# Autodesk Inventor assembly: spinning thing
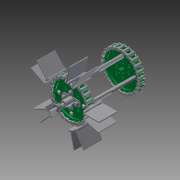
[picture p0: Inventor's stored thumbnail of the model, 180x180]
Saved by Autodesk Inventor 2014 SP1 (Build 180222100, 222)
## iProperties
Created: 2014-02-27
Part Number: spinning thing
Document SubType Name: Assembly
Designer: Ryan
Author: Ryan
## Documents named in this file (14)
- C:\Users\Ryan\Desktop\sw\toss up 5th A bot\intake\spinning thing.iam
- C:\Users\Ryan\Desktop\sw\lib\Aperture VEX CAD Library\Sprockets\HS Sprockets\High strength Chain Link.ipt
- C:\Users\Ryan\Desktop\sw\lib\Aperture VEX CAD Library\Tank Tread\flap-Link.ipt
- C:\Users\Ryan\Desktop\sw\lib\Aperture VEX CAD Library\Tank Tread\flaps\Conveyor-Fin-Tall.ipt
- C:\Users\Ryan\Desktop\sw\lib\Aperture VEX CAD Library\Sprockets\green\High Strength 24-Tooth Sprocket.ipt
- C:\Users\Ryan\Desktop\sw\lib\Aperture VEX CAD Library\Spacers\SPACER-0500-0375.ipt
- C:\Users\Ryan\Desktop\sw\lib\Aperture VEX CAD Library\Standoffs\BEAM-2000.ipt
- C:\Users\Ryan\Desktop\sw\lib\Aperture VEX CAD Library\Hardware\8-32\8-32_.375.ipt
- C:\Users\Ryan\Desktop\sw\lib\Aperture VEX CAD Library\Shaft\3 inch Shaft.ipt
- C:\Users\Ryan\Desktop\sw\lib\Aperture VEX CAD Library\Hardware\Shaft Collar.ipt
- C:\Users\Ryan\Desktop\sw\lib\Aperture VEX CAD Library\Sprockets\green\High Strength 24-Tooth Sprocket no knobs.ipt
- C:\Users\Ryan\Desktop\sw\lib\Aperture VEX CAD Library\Metal\Gussets\Lockbar.ipt
- C:\Users\Ryan\Desktop\sw\lib\Aperture VEX CAD Library\Hardware\8-32\8-32 nylock.ipt
- C:\Users\Ryan\Desktop\sw\lib\Aperture VEX CAD Library\Spacers\SPACER-0500-0250.ipt
## Components (91 placed, 13 different names)
1. High Strength 24-Tooth Sprocket no knobs:1 — Mate:15, Mate:16, Mate:17, Tangent:3, Mate:20, Mate:21, Mate:35, Mate:36, Flush:40, Mate:39, Mate:40, Mate:46, Mate:59, Mate:60, Tangent:8, Mate:66, Mate:67, Mate:69, Mate:70, Mate:78, Mate:79, Mate:80
2. SPACER-0500-0375:1 — Mate:18, Mate:43, Mate:44, Mate:73, Mate:84, Mate:85
3. High Strength 24-Tooth Sprocket:2 — Mate:25, Mate:26, Mate:33, Mate:34, Mate:37, Mate:38, Mate:18, Mate:72, Mate:48, Mate:61, Mate:62
4. 3 inch Shaft:1 — Flush:40, Mate:39, Mate:40, Mate:64, Mate:65, Mate:74
5. Shaft Collar:1 — Mate:71, Mate:72, Mate:73, Mate:74
6. Shaft Collar:2 — Mate:43, Mate:44
7. High strength Chain Link:35 — Mate:60
8. flap-Link:9 — Tangent:8
9. Conveyor-Fin-Tall:9
10. High strength Chain Link:36 — Flush:63, Mate:59, Mate:61
11. flap-Link:10 — Mate:62
12. Conveyor-Fin-Tall:10
13. Lockbar:1 — Mate:64, Mate:65, Mate:66, Mate:82, Mate:83
14. Lockbar:2 — Mate:67, Mate:69, Mate:70, Mate:71, Mate:75, Mate:76
15. SPACER-0500-0250:1 — Mate:83, Mate:84, Mate:85
16. flap-Link:2 — Mate:7, Mate:8, Mate:9, Mate:10, Flush:7, Mate:48
17. Conveyor-Fin-Tall:2 — Flush:8, Mate:11, Mate:12
18. flap-Link:1 — Mate:1, Mate:2, Mate:7, Flush:8, Mate:11, Mate:12, Tangent:3
19. High strength Chain Link:1 — Mate:1, Mate:2, Mate:8, Mate:13, Mate:14, Mate:17
20. High strength Chain Link:2 — Mate:13, Mate:14, Mate:15, Mate:16, Mate:45, Mate:47, Flush:63
21. High strength Chain Link:25 — Mate:45, Mate:46, Mate:47
22. Conveyor-Fin-Tall:1 — Mate:9, Mate:10, Flush:7
23. flap-Link:3
24. Conveyor-Fin-Tall:3
25. flap-Link:4
26. High strength Chain Link:26
27. High strength Chain Link:27
28. High strength Chain Link:28
29. Conveyor-Fin-Tall:6
30. flap-Link:5
31. Conveyor-Fin-Tall:4
32. flap-Link:6
33. High strength Chain Link:29
34. High strength Chain Link:30
35. High strength Chain Link:31
36. Conveyor-Fin-Tall:7
37. flap-Link:7
38. Conveyor-Fin-Tall:5
39. flap-Link:8
40. High strength Chain Link:32
41. High strength Chain Link:33
42. High strength Chain Link:34
43. Conveyor-Fin-Tall:8
44. 8-32_.375:11 — Mate:79, Mate:80, Mate:81
45. 8-32_.375:10 — Mate:75, Mate:76, Mate:77
46. 8-32 nylock:2 — Mate:81, Mate:82
47. 8-32 nylock:1 — Mate:77, Mate:78
48. 8-32_.375:12
49. 8-32_.375:13
50. 8-32 nylock:3
51. 8-32 nylock:4
52. BEAM-2000:1 — Mate:20, Mate:21, Mate:22, Mate:23
53. BEAM-2000:2 — Mate:22, Mate:23, Mate:25, Mate:26
54. 8-32_.375:3 — Mate:37, Mate:38
55. 8-32_.375:1 — Mate:35, Mate:36
56. BEAM-2000:3
57. BEAM-2000:4
58. 8-32_.375:14
59. 8-32_.375:15
60. BEAM-2000:5
61. BEAM-2000:6
62. 8-32_.375:16
63. 8-32_.375:17
64. BEAM-2000:7
65. BEAM-2000:8
66. 8-32_.375:18
67. 8-32_.375:19
68. High strength Chain Link:13 — Mate:33, Mate:34
69. High strength Chain Link:37
70. High strength Chain Link:38
71. High strength Chain Link:39
72. High strength Chain Link:40
73. High strength Chain Link:41
74. High strength Chain Link:42
75. High strength Chain Link:43
76. High strength Chain Link:44
77. High strength Chain Link:45
78. High strength Chain Link:46
79. High strength Chain Link:47
80. High strength Chain Link:48
81. High strength Chain Link:49
82. High strength Chain Link:50
83. High strength Chain Link:51
84. High strength Chain Link:52
85. High strength Chain Link:53
86. High strength Chain Link:54
87. High strength Chain Link:55
88. High strength Chain Link:56
89. High strength Chain Link:57
90. High strength Chain Link:58
91. High strength Chain Link:59
## Component patterns: (4 elements, first: flap-Link:2 + Conveyor-Fin-Tall:2 + flap-Link:1 + High strength Chain Link:1 + High strength Chain Link:2 + High strength Chain Link:25 + Conveyor-Fin-Tall:1), (2 elements, first: 8-32_.375:11 + 8-32_.375:10 + 8-32 nylock:2 + 8-32 nylock:1), (4 elements, first: BEAM-2000:1 + BEAM-2000:2 + 8-32_.375:3 + 8-32_.375:1), (24 elements, first: High strength Chain Link:13)
## Relationships (78: Mate 69, Flush 7, Tangent 2)
- Mate:1: flap-Link:1 ↔ High strength Chain Link:1
- Mate:2: flap-Link:1 ↔ High strength Chain Link:1
- [Flush]: High Strength 24-Tooth Sprocket no knobs:1 ↔ High strength Chain Link:1
- Mate:7: flap-Link:2 ↔ flap-Link:1
- Mate:8: flap-Link:2 ↔ High strength Chain Link:1
- Mate:9: flap-Link:2 ↔ Conveyor-Fin-Tall:1
- Mate:10: flap-Link:2 ↔ Conveyor-Fin-Tall:1
- Flush:7: flap-Link:2 ↔ Conveyor-Fin-Tall:1
- Flush:8: Conveyor-Fin-Tall:2 ↔ flap-Link:1
- Mate:11: Conveyor-Fin-Tall:2 ↔ flap-Link:1
- Mate:12: Conveyor-Fin-Tall:2 ↔ flap-Link:1
- Mate:13: High strength Chain Link:1 ↔ High strength Chain Link:2
- Mate:14: High strength Chain Link:1 ↔ High strength Chain Link:2
- Mate:15: High Strength 24-Tooth Sprocket no knobs:1 ↔ High strength Chain Link:2
- Mate:16: High Strength 24-Tooth Sprocket no knobs:1 ↔ High strength Chain Link:2
- Mate:17: High Strength 24-Tooth Sprocket no knobs:1 ↔ High strength Chain Link:1
- Tangent:3: High Strength 24-Tooth Sprocket no knobs:1 ↔ flap-Link:1
- Mate:18: SPACER-0500-0375:1 ↔ High Strength 24-Tooth Sprocket:2
- Mate:20: High Strength 24-Tooth Sprocket no knobs:1 ↔ BEAM-2000:1
- Mate:21: High Strength 24-Tooth Sprocket no knobs:1 ↔ BEAM-2000:1
- Mate:22: BEAM-2000:1 ↔ BEAM-2000:2
- Mate:23: BEAM-2000:1 ↔ BEAM-2000:2
- Mate:25: High Strength 24-Tooth Sprocket:2 ↔ BEAM-2000:2
- Mate:26: High Strength 24-Tooth Sprocket:2 ↔ BEAM-2000:2
- Mate:33: High Strength 24-Tooth Sprocket:2 ↔ High strength Chain Link:13
- Mate:34: High Strength 24-Tooth Sprocket:2 ↔ High strength Chain Link:13
- Mate:35: High Strength 24-Tooth Sprocket no knobs:1 ↔ 8-32_.375:1
- Mate:36: High Strength 24-Tooth Sprocket no knobs:1 ↔ 8-32_.375:1
- Mate:37: High Strength 24-Tooth Sprocket:2 ↔ 8-32_.375:3
- Mate:38: High Strength 24-Tooth Sprocket:2 ↔ 8-32_.375:3
- Flush:40 (29.2191 mm): High Strength 24-Tooth Sprocket no knobs:1 ↔ 3 inch Shaft:1
- Mate:39: High Strength 24-Tooth Sprocket no knobs:1 ↔ 3 inch Shaft:1
- Mate:40: High Strength 24-Tooth Sprocket no knobs:1 ↔ 3 inch Shaft:1
- Mate:43 (7.5184 mm): SPACER-0500-0375:1 ↔ Shaft Collar:2
- Mate:44: SPACER-0500-0375:1 ↔ Shaft Collar:2
- Mate:45: High strength Chain Link:2 ↔ High strength Chain Link:25
- Mate:46: High Strength 24-Tooth Sprocket no knobs:1 ↔ High strength Chain Link:25
- Mate:47: High strength Chain Link:2 ↔ High strength Chain Link:25
- Mate:48 (37.5412 mm): High Strength 24-Tooth Sprocket:2 ↔ flap-Link:2
- [Mate]: High strength Chain Link:35 ↔ flap-Link:9
- [Mate]: High strength Chain Link:35 ↔ flap-Link:9
- [Mate]: flap-Link:9 ↔ flap-Link:10
- [Mate]: High strength Chain Link:35 ↔ flap-Link:10
- [Mate]: Conveyor-Fin-Tall:9 ↔ flap-Link:10
- [Mate]: Conveyor-Fin-Tall:9 ↔ flap-Link:10
- [Flush]: Conveyor-Fin-Tall:9 ↔ flap-Link:10
- [Flush]: flap-Link:9 ↔ Conveyor-Fin-Tall:10
- [Mate]: flap-Link:9 ↔ Conveyor-Fin-Tall:10
- [Mate]: flap-Link:9 ↔ Conveyor-Fin-Tall:10
- [Mate]: High strength Chain Link:35 ↔ High strength Chain Link:36
- [Mate]: High strength Chain Link:35 ↔ High strength Chain Link:36
- Flush:63: High strength Chain Link:36 ↔ High strength Chain Link:2
- Mate:59: High Strength 24-Tooth Sprocket no knobs:1 ↔ High strength Chain Link:36
- Mate:60: High Strength 24-Tooth Sprocket no knobs:1 ↔ High strength Chain Link:35
- Tangent:8: High Strength 24-Tooth Sprocket no knobs:1 ↔ flap-Link:9
- Mate:61 (37.5412 mm): High Strength 24-Tooth Sprocket:2 ↔ High strength Chain Link:36
- Mate:62 (37.6428 mm): High Strength 24-Tooth Sprocket:2 ↔ flap-Link:10
- Mate:64: 3 inch Shaft:1 ↔ Lockbar:1
- Mate:65: 3 inch Shaft:1 ↔ Lockbar:1
- Mate:66: High Strength 24-Tooth Sprocket no knobs:1 ↔ Lockbar:1
- Mate:67: High Strength 24-Tooth Sprocket no knobs:1 ↔ Lockbar:2
- Mate:69: High Strength 24-Tooth Sprocket no knobs:1 ↔ Lockbar:2
- Mate:70: High Strength 24-Tooth Sprocket no knobs:1 ↔ Lockbar:2
- Mate:71: Shaft Collar:1 ↔ Lockbar:2
- Mate:72: High Strength 24-Tooth Sprocket:2 ↔ Shaft Collar:1
- Mate:73: SPACER-0500-0375:1 ↔ Shaft Collar:1
- Mate:74 (-1.5875 mm): 3 inch Shaft:1 ↔ Shaft Collar:1
- Mate:75: Lockbar:2 ↔ 8-32_.375:10
- Mate:76: Lockbar:2 ↔ 8-32_.375:10
- Mate:77: 8-32_.375:10 ↔ 8-32 nylock:1
- Mate:78: High Strength 24-Tooth Sprocket no knobs:1 ↔ 8-32 nylock:1
- Mate:79: High Strength 24-Tooth Sprocket no knobs:1 ↔ 8-32_.375:11
- Mate:80: High Strength 24-Tooth Sprocket no knobs:1 ↔ 8-32_.375:11
- Mate:81: 8-32_.375:11 ↔ 8-32 nylock:2
- Mate:82: Lockbar:1 ↔ 8-32 nylock:2
- Mate:83: Lockbar:1 ↔ SPACER-0500-0250:1
- Mate:84: SPACER-0500-0375:1 ↔ SPACER-0500-0250:1
- Mate:85: SPACER-0500-0375:1 ↔ SPACER-0500-0250:1
## Named parameters: d79_d15 = 0 mm, d80_d16 = 0 mm, d81_d17 = 0 mm, d82_d18 = 0 mm, d83_d19 = 0 mm, d84_d20 = 0 mm, d85_d23 = 0 mm, d86_d24 = 0 mm, d87_d0 = 0 mm, d88_d1 = 0 mm, d89_d10 = 0 mm, d90_d11 = 0 mm
